# Autodesk Inventor assembly: PIANO HINGE
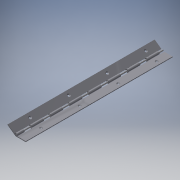
[picture p0: Inventor's stored thumbnail of the model, 180x180]
Saved by Autodesk Inventor 2016 (Build 200138000, 138)
## iProperties
Created: 2015-09-17
Part Number: PIANO HINGE
Document SubType Name: Assembly
Designer: testing
Author: testing
## Documents named in this file (4)
- \\Mac\Home\Desktop\1510-stronghold-CAD-master\chassis\request-piano-hinge-1\PIANO HINGE.iam
- \\Mac\Home\Desktop\1510-stronghold-CAD-master\chassis\request-piano-hinge-1\SIDE 1.ipt
- \\Mac\Home\Desktop\1510-stronghold-CAD-master\chassis\request-piano-hinge-1\SIDE 2.ipt
- \\Mac\Home\Desktop\1510-stronghold-CAD-master\chassis\request-piano-hinge-1\PIVOT WIRE.ipt
## Components (3 placed, 3 different names)
1. SIDE 1:1 — Mate:1, Flush:1, Flush:2, Mate:2
2. SIDE 2:1 — Flush:2, Mate:2
3. PIVOT WIRE:1 — Mate:1, Flush:1
## Relationships (4: Mate 2, Flush 2)
- Mate:1: SIDE 1:1 ↔ PIVOT WIRE:1
- Flush:1: SIDE 1:1 ↔ PIVOT WIRE:1
- Flush:2: SIDE 1:1 ↔ SIDE 2:1
- Mate:2: SIDE 1:1 ↔ SIDE 2:1
